# Autodesk Inventor assembly: GP9-100
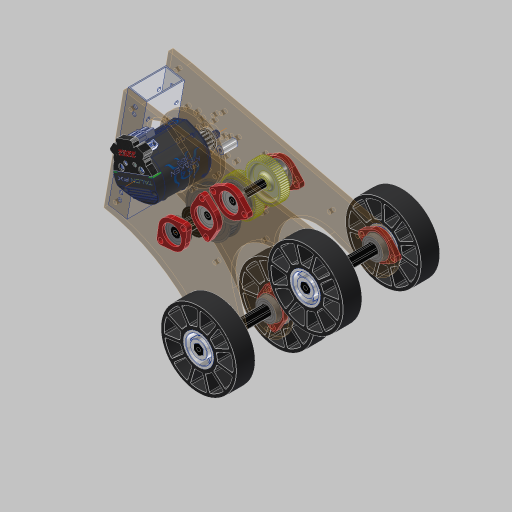
[picture p0: Inventor's stored thumbnail of the model, 512x512]
Saved by Autodesk Inventor 2023.5 (Build 275446000, 446)
## iProperties
Created: 2025-02-27
Part Number: GP9-100
Document SubType Name: Assembly
Designer: dlangdon
Author: dlangdon
## Documents named in this file (23)
- C:\Users\slick\OneDrive\Desktop\2025-ReefScape---CAD\Gripper\GP9\GP9-100.iam
- C:\Users\slick\OneDrive\Desktop\2025-ReefScape---CAD\Gripper\GP9\GP9-001.ipt
- C:\Users\slick\OneDrive\Desktop\2025-ReefScape---CAD\Gripper\GP9\GP9-002.ipt
- C:\Users\slick\OneDrive\Desktop\2025-ReefScape---CAD\Gripper\GP9\GP9-004.ipt
- C:\Users\slick\OneDrive\Desktop\2025-ReefScape---CAD\Gripper\GP9\GP9-003.ipt
- C:\Users\slick\OneDrive\Desktop\2025-ReefScape---CAD\Gripper\GP6\GP6-006.ipt
- C:\Users\slick\OneDrive\Desktop\2025-ReefScape---CAD\COMMON PARTS\MOTORS\Kracken with Cover and Boards.iam
- C:\Users\slick\OneDrive\Desktop\2025-ReefScape---CAD\COMMON PARTS\WHEELS\am-3480 4IN 500Hex Bore Compliant Wheel REV2 (1).iam
- C:\Users\slick\OneDrive\Desktop\2025-ReefScape---CAD\Field Items\Game Pieces\GE-25500.ipt
- C:\Users\slick\OneDrive\Desktop\2025-ReefScape---CAD\Field Items\Game Pieces\GE-25501.ipt
- C:\Users\slick\OneDrive\Desktop\2025-ReefScape---CAD\COMMON PARTS\PULLEYS\htd\36t_x_9mm_Wide_Double_Flange_Aluminum_Pulley_HTD_5mm_1_2_Hex_Bore_217-3231.ipt
- C:\Users\slick\OneDrive\Desktop\2025-ReefScape---CAD\COMMON PARTS\PULLEYS\htd\WCP-1017 (1)\WCP-1017 (1).ipt
- C:\Users\slick\OneDrive\Desktop\2025-ReefScape---CAD\COMMON PARTS\PULLEYS\htd\18t_x_9mm_Wide_Double_Flange_Aluminum_Pulley_HTD_5mm_1_2_Hex_Bore_217-3225.ipt
- C:\Users\slick\OneDrive\Desktop\2025-ReefScape---CAD\COMMON PARTS\PULLEYS\htd\24t_x_9mm_Wide_Double_Flange_Aluminum_Pulley_HTD_5mm_1_2_Hex_Bore_217-3227.ipt
- C:\Users\slick\OneDrive\Desktop\2025-ReefScape---CAD\COMMON PARTS\GEARS\32 dp gear\60t_Aluminum_Spur_Gear_32_DP_3_8_Hex_Bore_217-5863.ipt
- C:\Users\slick\OneDrive\Desktop\2025-ReefScape---CAD\COMMON PARTS\BEARINGS\13_75mm_1_2_ThunderHex_ID_x_1_125_OD_x_0_313_WD_Flanged_Bearing_217-4006.ipt
- C:\Users\slick\OneDrive\Desktop\2025-ReefScape---CAD\COMMON PARTS\BEARINGS\0_500_ID_x_1_125_OD_x_0_313_WD_Flanged_Bearing_217-2731.ipt
- C:\Users\slick\OneDrive\Desktop\2025-ReefScape---CAD\COMMON PARTS\BEARINGS\Bearing Retainer\Retainer.ipt
- C:\Users\slick\OneDrive\Desktop\2025-ReefScape---CAD\Gripper\GP9\GP9-005.ipt
- C:\Users\slick\OneDrive\Desktop\2025-ReefScape---CAD\Gripper\GP9\GP9-006.ipt
- C:\Users\slick\OneDrive\Desktop\2025-ReefScape---CAD\COMMON PARTS\BEARINGS\0_375_ID_x_1_125_OD_x_0_313_WD_Flanged_Bearing_217-2732.ipt
- C:\Users\slick\OneDrive\Desktop\2025-ReefScape---CAD\Gripper\GP9\GP9-007.ipt
- C:\Users\slick\OneDrive\Desktop\2025-ReefScape---CAD\Gripper\GP9\GP9-008.ipt
## Components (48 placed, 22 different names)
1. GP9-001:1 — Insert:7, Insert:8, Mate:1, Mate:4, Insert:14, Insert:15, Insert:18, Insert:19, Insert:24, Insert:34, Insert:35, Insert:36, Insert:37, Insert:38, Insert:39, Insert:40, Insert:41, Insert:42, Insert:43, Insert:53, Insert:55
2. GP9-002:1 — Mate:2, Mate:3, Mate:5, Insert:12, Insert:13, Insert:16, Insert:17, Insert:25, Insert:26, Insert:27, Insert:28, Insert:29, Insert:30, Insert:31, Insert:32, Insert:33, Insert:47, Insert:48, Insert:52, Insert:54
3. GP9-004:1 — Insert:12, Insert:13, Insert:14, Insert:15
4. GP9-003:1 — Insert:5, Insert:6, Insert:10, Insert:11, Mate:7
5. GP6-006:1 — Insert:6, Insert:7
6. GP6-006:2 — Insert:5, Insert:8
7. Kracken with Cover and Boards:1 [sub-assembly] — Insert:10, Insert:11, Mate:6
8. am-3480 4IN 500Hex Bore Compliant Wheel REV2 (1):1 [sub-assembly] — Mate:3, Flush:1, Mate:15, Insert:50
9. am-3480 4IN 500Hex Bore Compliant Wheel REV2 (1):2 [sub-assembly] — Mate:2, Flush:1, Insert:51
10. am-3480 4IN 500Hex Bore Compliant Wheel REV2 (1):3 [sub-assembly] — Mate:1, Flush:2
11. am-3480 4IN 500Hex Bore Compliant Wheel REV2 (1):4 [sub-assembly] — Mate:4, Flush:2, Mate:16
12. GE-25500:1 — Mate:5
13. GE-25501:1
14. WCP-1017 (1):1 — Mate:6, Mate:7, Flush:3
15. 18t_x_9mm_Wide_Double_Flange_Aluminum_Pulley_HTD_5mm_1_2_Hex_Bore_217-3225:1 — Mate:13, Flush:4
16. 36t_x_9mm_Wide_Double_Flange_Aluminum_Pulley_HTD_5mm_1_2_Hex_Bore_217-3231:2 — Mate:12, Flush:3
17. 24t_x_9mm_Wide_Double_Flange_Aluminum_Pulley_HTD_5mm_1_2_Hex_Bore_217-3227:1 — Flush:4
18. 60t_Aluminum_Spur_Gear_32_DP_3_8_Hex_Bore_217-5863:1 — Flush:5
19. 13_75mm_1_2_ThunderHex_ID_x_1_125_OD_x_0_313_WD_Flanged_Bearing_217-4006:1 — Insert:17, Insert:44
20. 13_75mm_1_2_ThunderHex_ID_x_1_125_OD_x_0_313_WD_Flanged_Bearing_217-4006:2 — Insert:16, Insert:46
21. 13_75mm_1_2_ThunderHex_ID_x_1_125_OD_x_0_313_WD_Flanged_Bearing_217-4006:3 — Insert:18, Insert:45
22. 13_75mm_1_2_ThunderHex_ID_x_1_125_OD_x_0_313_WD_Flanged_Bearing_217-4006:4 — Insert:19, Insert:49
23. 0_375_ID_x_1_125_OD_x_0_313_WD_Flanged_Bearing_217-2732:3 — Insert:53
24. 0_375_ID_x_1_125_OD_x_0_313_WD_Flanged_Bearing_217-2732:4 — Insert:52, Insert:57
25. 0_375_ID_x_1_125_OD_x_0_313_WD_Flanged_Bearing_217-2732:5 — Insert:55
26. 0_375_ID_x_1_125_OD_x_0_313_WD_Flanged_Bearing_217-2732:6 — Insert:54, Insert:58
27. 0_500_ID_x_1_125_OD_x_0_313_WD_Flanged_Bearing_217-2731:1 — Insert:25, Insert:56
28. 0_500_ID_x_1_125_OD_x_0_313_WD_Flanged_Bearing_217-2731:2 — Insert:24, Mate:12, Mate:13
29. Retainer:1 — Insert:26, Insert:27
30. Retainer:2 — Insert:28, Insert:29
31. Retainer:4 — Insert:30, Insert:31
32. Retainer:5 — Insert:32, Insert:33
33. Retainer:6 — Insert:47, Insert:48
34. Retainer:7 — Insert:34, Insert:35
35. Retainer:8 — Insert:36, Insert:37
36. Retainer:10 — Insert:42, Insert:43
37. Retainer:11 — Insert:40, Insert:41
38. Retainer:12 — Insert:38, Insert:39
39. GP9-005:1 — Insert:49, Mate:16
40. GP9-005:2 — Insert:45
41. GP9-005:3 — Insert:46, Mate:15
42. GP9-005:4 — Insert:44
43. 60t_Aluminum_Spur_Gear_32_DP_3_8_Hex_Bore_217-5863:2 — Flush:5
44. GP9-006:1 — Insert:50
45. GP9-006:2 — Insert:51
46. GP9-007:1 — Insert:56
47. GP9-008:1 — Insert:57
48. GP9-008:2 — Insert:58
## Relationships (68: Insert 49, Mate 14, Flush 5)
- Insert:5: GP9-003:1 ↔ GP6-006:2
- Insert:6: GP9-003:1 ↔ GP6-006:1
- Insert:7: GP9-001:1 ↔ GP6-006:1
- Insert:8: GP9-001:1 ↔ GP6-006:2
- Insert:10: GP9-003:1 ↔ Kracken with Cover and Boards:1
- Insert:11: GP9-003:1 ↔ Kracken with Cover and Boards:1
- Mate:1: GP9-001:1 ↔ am-3480 4IN 500Hex Bore Compliant Wheel REV2 (1):3
- Mate:2: GP9-002:1 ↔ am-3480 4IN 500Hex Bore Compliant Wheel REV2 (1):2
- Mate:3: GP9-002:1 ↔ am-3480 4IN 500Hex Bore Compliant Wheel REV2 (1):1
- Mate:4: GP9-001:1 ↔ am-3480 4IN 500Hex Bore Compliant Wheel REV2 (1):4
- Flush:1: am-3480 4IN 500Hex Bore Compliant Wheel REV2 (1):1 ↔ am-3480 4IN 500Hex Bore Compliant Wheel REV2 (1):2
- Flush:2: am-3480 4IN 500Hex Bore Compliant Wheel REV2 (1):3 ↔ am-3480 4IN 500Hex Bore Compliant Wheel REV2 (1):4
- Mate:5: GP9-002:1 ↔ GE-25500:1
- Insert:12: GP9-002:1 ↔ GP9-004:1
- Insert:13: GP9-002:1 ↔ GP9-004:1
- Insert:14: GP9-001:1 ↔ GP9-004:1
- Insert:15: GP9-001:1 ↔ GP9-004:1
- Insert:16: GP9-002:1 ↔ 13_75mm_1_2_ThunderHex_ID_x_1_125_OD_x_0_313_WD_Flanged_Bearing_217-4006:2
- Insert:17: GP9-002:1 ↔ 13_75mm_1_2_ThunderHex_ID_x_1_125_OD_x_0_313_WD_Flanged_Bearing_217-4006:1
- Insert:18: GP9-001:1 ↔ 13_75mm_1_2_ThunderHex_ID_x_1_125_OD_x_0_313_WD_Flanged_Bearing_217-4006:3
- Insert:19: GP9-001:1 ↔ 13_75mm_1_2_ThunderHex_ID_x_1_125_OD_x_0_313_WD_Flanged_Bearing_217-4006:4
- Insert:24: GP9-001:1 ↔ 0_500_ID_x_1_125_OD_x_0_313_WD_Flanged_Bearing_217-2731:2
- Insert:25: GP9-002:1 ↔ 0_500_ID_x_1_125_OD_x_0_313_WD_Flanged_Bearing_217-2731:1
- Insert:26: GP9-002:1 ↔ Retainer:1
- Insert:27: GP9-002:1 ↔ Retainer:1
- Insert:28: GP9-002:1 ↔ Retainer:2
- Insert:29: GP9-002:1 ↔ Retainer:2
- Insert:30: GP9-002:1 ↔ Retainer:4
- Insert:31: GP9-002:1 ↔ Retainer:4
- Insert:32: GP9-002:1 ↔ Retainer:5
- Insert:33: GP9-002:1 ↔ Retainer:5
- Insert:34: GP9-001:1 ↔ Retainer:7
- Insert:35: GP9-001:1 ↔ Retainer:7
- Insert:36: GP9-001:1 ↔ Retainer:8
- Insert:37: GP9-001:1 ↔ Retainer:8
- Insert:38: GP9-001:1 ↔ Retainer:12
- Insert:39: GP9-001:1 ↔ Retainer:12
- Insert:40: GP9-001:1 ↔ Retainer:11
- Insert:41: GP9-001:1 ↔ Retainer:11
- Insert:42: GP9-001:1 ↔ Retainer:10
- Insert:43: GP9-001:1 ↔ Retainer:10
- Insert:44: 13_75mm_1_2_ThunderHex_ID_x_1_125_OD_x_0_313_WD_Flanged_Bearing_217-4006:1 ↔ GP9-005:4
- Insert:45: 13_75mm_1_2_ThunderHex_ID_x_1_125_OD_x_0_313_WD_Flanged_Bearing_217-4006:3 ↔ GP9-005:2
- Insert:46: 13_75mm_1_2_ThunderHex_ID_x_1_125_OD_x_0_313_WD_Flanged_Bearing_217-4006:2 ↔ GP9-005:3
- Insert:47: GP9-002:1 ↔ Retainer:6
- Insert:48: GP9-002:1 ↔ Retainer:6
- Insert:49: 13_75mm_1_2_ThunderHex_ID_x_1_125_OD_x_0_313_WD_Flanged_Bearing_217-4006:4 ↔ GP9-005:1
- Mate:6: Kracken with Cover and Boards:1 ↔ WCP-1017 (1):1
- Mate:7: GP9-003:1 ↔ WCP-1017 (1):1
- [Mate]: 24t_x_9mm_Wide_Double_Flange_Aluminum_Pulley_HTD_5mm_1_2_Hex_Bore_217-3227:1 ↔ 0_375_ID_x_1_125_OD_x_0_313_WD_Flanged_Bearing_217-2732:3
- [Mate]: 60t_Aluminum_Spur_Gear_32_DP_3_8_Hex_Bore_217-5863:1 ↔ 0_375_ID_x_1_125_OD_x_0_313_WD_Flanged_Bearing_217-2732:3
- Mate:12: 36t_x_9mm_Wide_Double_Flange_Aluminum_Pulley_HTD_5mm_1_2_Hex_Bore_217-3231:2 ↔ 0_500_ID_x_1_125_OD_x_0_313_WD_Flanged_Bearing_217-2731:2
- Mate:13: 18t_x_9mm_Wide_Double_Flange_Aluminum_Pulley_HTD_5mm_1_2_Hex_Bore_217-3225:1 ↔ 0_500_ID_x_1_125_OD_x_0_313_WD_Flanged_Bearing_217-2731:2
- Flush:3: WCP-1017 (1):1 ↔ 36t_x_9mm_Wide_Double_Flange_Aluminum_Pulley_HTD_5mm_1_2_Hex_Bore_217-3231:2
- Flush:4: 18t_x_9mm_Wide_Double_Flange_Aluminum_Pulley_HTD_5mm_1_2_Hex_Bore_217-3225:1 ↔ 24t_x_9mm_Wide_Double_Flange_Aluminum_Pulley_HTD_5mm_1_2_Hex_Bore_217-3227:1
- [Mate]: 0_375_ID_x_1_125_OD_x_0_313_WD_Flanged_Bearing_217-2732:5 ↔ 60t_Aluminum_Spur_Gear_32_DP_3_8_Hex_Bore_217-5863:2
- Flush:5: 60t_Aluminum_Spur_Gear_32_DP_3_8_Hex_Bore_217-5863:1 ↔ 60t_Aluminum_Spur_Gear_32_DP_3_8_Hex_Bore_217-5863:2
- Mate:15: am-3480 4IN 500Hex Bore Compliant Wheel REV2 (1):1 ↔ GP9-005:3
- Mate:16: am-3480 4IN 500Hex Bore Compliant Wheel REV2 (1):4 ↔ GP9-005:1
- Insert:50: am-3480 4IN 500Hex Bore Compliant Wheel REV2 (1):1 ↔ GP9-006:1
- Insert:51: am-3480 4IN 500Hex Bore Compliant Wheel REV2 (1):2 ↔ GP9-006:2
- Insert:52: GP9-002:1 ↔ 0_375_ID_x_1_125_OD_x_0_313_WD_Flanged_Bearing_217-2732:4
- Insert:53: GP9-001:1 ↔ 0_375_ID_x_1_125_OD_x_0_313_WD_Flanged_Bearing_217-2732:3
- Insert:54: GP9-002:1 ↔ 0_375_ID_x_1_125_OD_x_0_313_WD_Flanged_Bearing_217-2732:6
- Insert:55: GP9-001:1 ↔ 0_375_ID_x_1_125_OD_x_0_313_WD_Flanged_Bearing_217-2732:5
- Insert:56: 0_500_ID_x_1_125_OD_x_0_313_WD_Flanged_Bearing_217-2731:1 ↔ GP9-007:1
- Insert:57: 0_375_ID_x_1_125_OD_x_0_313_WD_Flanged_Bearing_217-2732:4 ↔ GP9-008:1
- Insert:58: 0_375_ID_x_1_125_OD_x_0_313_WD_Flanged_Bearing_217-2732:6 ↔ GP9-008:2
